# Autodesk Inventor assembly: Montagem Ze Guia
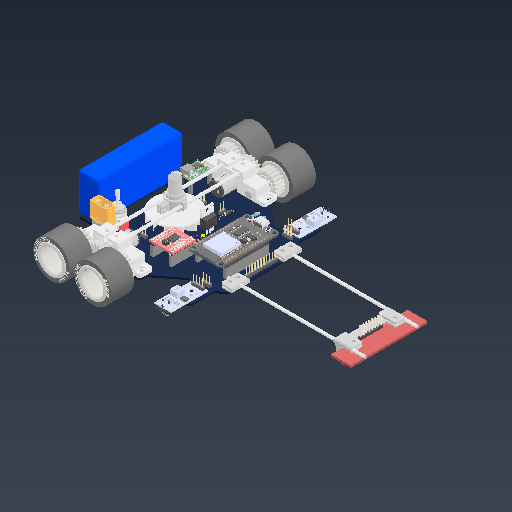
[picture p0: Inventor's stored thumbnail of the model, 512x512]
Saved by Autodesk Inventor 2026.1 (Build 301233020, 233B)
## iProperties
Created: 2026-02-13
Part Number: Montagem Ze Guia
Document SubType Name: Assembly
Designer: celio
Author: celio
## Documents named in this file (23)
- C:\Users\celio\OneDrive\Documentos\Inventor\ZeGuia\Montagem Ze Guia.iam
- C:\Users\celio\OneDrive\Documentos\Inventor\ZeGuia\Placa\PCB.ipt
- C:\Users\celio\OneDrive\Documentos\Inventor\ZeGuia\Bateria\Bateria.ipt
- C:\Users\celio\OneDrive\Documentos\Inventor\ZeGuia\Montagem\4x2\Base\4x2.iam
- C:\Users\celio\OneDrive\Documentos\Inventor\ZeGuia\Montagem\Turbina\Turbina.iam
- C:\Users\celio\OneDrive\Documentos\Inventor\ZeGuia\Sensores\TCRT5000\TCRT5000.iam
- C:\Users\celio\OneDrive\Documentos\Inventor\ZeGuia\Componentes\Controlador\esp32\esp32_30pin.iam
- C:\Users\celio\OneDrive\Documentos\Inventor\ZeGuia\Componentes\Ponte H\TB6612FNG\TB6612FNG.iam
- C:\Users\celio\OneDrive\Documentos\Inventor\ZeGuia\Sensores\QTR8RC\Qtr-8RC.ipt
- C:\Users\celio\OneDrive\Documentos\Inventor\ZeGuia\Pinos\Macho\1x11\1x11.iam
- C:\Users\celio\OneDrive\Documentos\Inventor\ZeGuia\Componentes\Regulador\Mini - 360.iam
- C:\Users\celio\OneDrive\Documentos\Inventor\ZeGuia\Componentes\Eletronica\Diodo\Diodo 1N4007.ipt
- C:\Users\celio\OneDrive\Documentos\Inventor\ZeGuia\Pinos\Macho\1x2\1x2.iam
- C:\Users\celio\OneDrive\Documentos\Inventor\ZeGuia\Componentes\Eletronica\MOSFET\irlz44n.ipt
- C:\Users\celio\OneDrive\Documentos\Inventor\ZeGuia\Componentes\Switch\SPDT Toggle Switch.iam
- C:\Users\celio\OneDrive\Documentos\Inventor\ZeGuia\Bateria\Conector XT60\XT60.iam
- C:\Users\celio\OneDrive\Documentos\Inventor\ZeGuia\Componentes\Eletronica\Resistor\RES-0.25W-H-MF.ipt
- C:\Users\celio\OneDrive\Documentos\Inventor\ZeGuia\Componentes\Eletronica\Capacitor\Ceramico\CAP_DISC_4x3_YL.ipt
- C:\Users\celio\OneDrive\Documentos\Inventor\ZeGuia\Componentes\Eletronica\Capacitor\Eletrolitico\CAP_RAD_D8x15_POL_BK.ipt
- C:\Users\celio\OneDrive\Documentos\Inventor\ZeGuia\Pinos\Macho\1x3\1x3.iam
- C:\Users\celio\OneDrive\Documentos\Inventor\ZeGuia\3D\Suporte\Haste sensor\Sup_haste_corpo.ipt
- C:\Users\celio\OneDrive\Documentos\Inventor\ZeGuia\3D\Suporte\HASTE_FIBRA.ipt
- C:\Users\celio\OneDrive\Documentos\Inventor\ZeGuia\3D\Suporte\Haste sensor\Sup_haste_sensor.iam
## Components (36 placed, 22 different names)
1. PCB:1 — Coincidente:1, Coincidente:2, Coincidente:3, Alinhado:1, Coincidente:4, Coincidente:5, Coincidente:6, Coincidente:7, Coincidente:9, Coincidente:10, Coincidente:11, Coincidente:12, Coincidente:13, Coincidente:14, Coincidente:15, Coincidente:16, Coincidente:17, Alinhado:2, Alinhado:3, Coincidente:18, Coincidente:19
2. Bateria:1 — Coincidente:1
3. 4x2:1 [sub-assembly] — Coincidente:3, Coincidente:20
4. 4x2:2 [sub-assembly] — Coincidente:2, Alinhado:2, Alinhado:3, Coincidente:21
5. Turbina:1 [sub-assembly] — Alinhado:1
6. TCRT5000:1 [sub-assembly] — Coincidente:4
7. TCRT5000:2 [sub-assembly] — Coincidente:5
8. esp32_30pin:1 [sub-assembly] — Coincidente:6
9. TB6612FNG:1 [sub-assembly] — Coincidente:7
10. Qtr-8RC:1 — Coincidente:10
11. 1x11:1 [sub-assembly] — Coincidente:9
12. Mini - 360:1 [sub-assembly] — Coincidente:11
13. Diodo 1N4007:1
14. 1x2:1 [sub-assembly] — Coincidente:12
15. irlz44n:1
16. SPDT Toggle Switch:1 [sub-assembly] — Coincidente:13
17. XT60:1 [sub-assembly]
18. RES-0.25W-H-MF:1
19. RES-0.25W-H-MF:2
20. RES-0.25W-H-MF:3
21. RES-0.25W-H-MF:4
22. CAP_DISC_4x3_YL:1
23. CAP_RAD_D8x15_POL_BK:1
24. CAP_DISC_4x3_YL:2
25. CAP_DISC_4x3_YL:3
26. 1x2:2 [sub-assembly] — Coincidente:14
27. 1x2:3 [sub-assembly] — Coincidente:15
28. 1x3:1 [sub-assembly] — Coincidente:16
29. 1x3:2 [sub-assembly] — Coincidente:17
30. Sup_haste_corpo:1 — Coincidente:18
31. Sup_haste_corpo:2 — Coincidente:19
32. HASTE_FIBRA:1
33. HASTE_FIBRA:2
34. HASTE_FIBRA:3 — Coincidente:21
35. HASTE_FIBRA:4 — Coincidente:20
36. Sup_haste_sensor:1 [sub-assembly]
## Relationships (24: Mate 20, Flush 4)
- Coincidente:1 [Mate]: PCB:1 ↔ Bateria:1
- Coincidente:2 [Mate]: PCB:1 ↔ 4x2:2
- Coincidente:3 [Mate]: PCB:1 ↔ 4x2:1
- Alinhado:1 [Flush] (-8 mm): PCB:1 ↔ Turbina:1
- Coincidente:4 [Mate]: PCB:1 ↔ TCRT5000:1
- Coincidente:5 [Mate]: PCB:1 ↔ TCRT5000:2
- Coincidente:6 [Mate] (11 mm): PCB:1 ↔ esp32_30pin:1
- Coincidente:7 [Mate] (10 mm): PCB:1 ↔ TB6612FNG:1
- Coincidente:9 [Mate]: PCB:1 ↔ 1x11:1
- Coincidente:10 [Mate] (-1.6 mm): PCB:1 ↔ Qtr-8RC:1
- Coincidente:11 [Mate] (10 mm): PCB:1 ↔ Mini - 360:1
- Coincidente:12 [Mate]: PCB:1 ↔ 1x2:1
- Coincidente:13 [Mate]: PCB:1 ↔ SPDT Toggle Switch:1
- Coincidente:14 [Mate]: PCB:1 ↔ 1x2:2
- Coincidente:15 [Mate]: PCB:1 ↔ 1x2:3
- Coincidente:16 [Mate]: PCB:1 ↔ 1x3:1
- Coincidente:17 [Mate]: PCB:1 ↔ 1x3:2
- Alinhado:2 [Flush]: PCB:1 ↔ 4x2:2
- Alinhado:3 [Flush]: PCB:1 ↔ 4x2:2
- Coincidente:18 [Mate]: PCB:1 ↔ Sup_haste_corpo:1
- Coincidente:19 [Mate]: PCB:1 ↔ Sup_haste_corpo:2
- Alinhado:4 [Flush] (-10.5 mm)
- Coincidente:20 [Mate]: 4x2:1 ↔ HASTE_FIBRA:4
- Coincidente:21 [Mate]: 4x2:2 ↔ HASTE_FIBRA:3
